# Autodesk Inventor assembly: SpMax_Drive
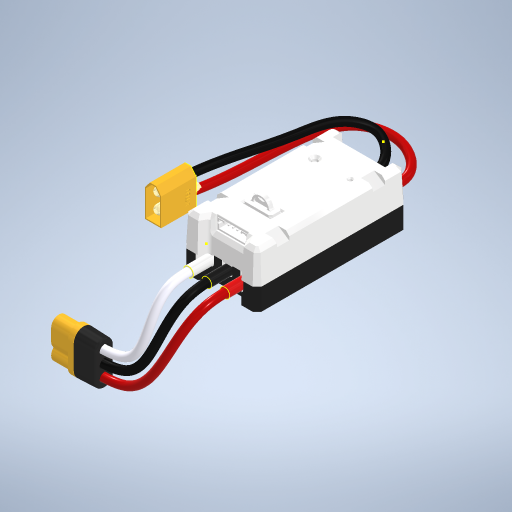
[picture p0: Inventor's stored thumbnail of the model, 512x512]
Saved by Autodesk Inventor 2023 (Build 270158000, 158)
## iProperties
Created: 2023-09-14
Part Number: SpMax_Drive
Document SubType Name: Assembly
Designer: adamarnold
Author: adamarnold
## Documents named in this file (5)
- I:\My Drive\1939\2_Design\2023-2024\Parts\Electronics\SpMax_Drive.iam
- I:\My Drive\1939\2_Design\2023-2024\Parts\Electronics\REV-11-2158-Spark-MAX_Wired.ipt
- I:\My Drive\1939\2_Design\2023-2024\Parts\Electronics\Connectors\XT60_Recp.ipt
- I:\My Drive\1939\2_Design\2023-2024\Parts\Electronics\Component Wiring\SPM_Power_Phase_Wiring.iam
- I:\My Drive\1939\2_Design\2023-2024\Parts\Electronics\Connectors\MR60_Plug.iam
## Components (4 placed, 4 different names)
1. REV-11-2158-Spark-MAX_Wired:1 — Mate:1, Flush:1, Mate:2, Flush:2, Flush:3, Mate:3, Mate:4, Flush:4, Mate:5
2. XT60_Recp:1 — Flush:2, Flush:3, Mate:3
3. MR60_Plug:1 [sub-assembly] — Mate:4, Flush:4, Mate:5
4. SPM_Power_Phase_Wiring [sub-assembly]
## Relationships (9: Mate 5, Flush 4)
- Mate:1: REV-11-2158-Spark-MAX_Wired:1
- Flush:1: REV-11-2158-Spark-MAX_Wired:1
- Mate:2: REV-11-2158-Spark-MAX_Wired:1
- Flush:2 (12.7 mm): REV-11-2158-Spark-MAX_Wired:1 ↔ XT60_Recp:1
- Flush:3: REV-11-2158-Spark-MAX_Wired:1 ↔ XT60_Recp:1
- Mate:3 (9.525 mm): REV-11-2158-Spark-MAX_Wired:1 ↔ XT60_Recp:1
- Mate:4 (16.0274 mm): REV-11-2158-Spark-MAX_Wired:1 ↔ MR60_Plug:1
- Flush:4 (66.294 mm): REV-11-2158-Spark-MAX_Wired:1 ↔ MR60_Plug:1
- Mate:5 (38.1 mm): REV-11-2158-Spark-MAX_Wired:1 ↔ MR60_Plug:1
